# Autodesk Inventor assembly: Turnigy SK8 5045 (IGES V1)
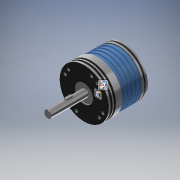
[picture p0: Inventor's stored thumbnail of the model, 180x180]
Saved by Autodesk Inventor 2019.2 (Build 232265000, 265)
## iProperties
Company: unknown
Created: 2018-11-25
Part Number: Turnigy SK8 5045 (IGES V1)
Document SubType Name: Assembly
Designer: Petar
Sending System: unknown
Preprocessor: unknown
Minimum Resolution: 0.01
Sending System Product ID: Turnigy SK8 5045 (IGES V1)
Sent Units: Millimeter
Translation Standard: IGES 5.3
Model Creation Time: 2018-11-25
Title: Turnigy SK8 5045 (IGES V1)
Author: emisnug
## Documents named in this file (8)
- D:\OMG\E-Board\CAD\Inventor\Electric Motor\Turnigy SK8 5045 (IGES V1).iam
- D:\OMG\E-Board\CAD\Inventor\Electric Motor\Magnets v9.ipt
- D:\OMG\E-Board\CAD\Inventor\Electric Motor\Can v14.ipt
- D:\OMG\E-Board\CAD\Inventor\Electric Motor\Shaft v2.ipt
- D:\OMG\E-Board\CAD\Inventor\Electric Motor\Stator Core v1.ipt
- D:\OMG\E-Board\CAD\Inventor\Electric Motor\Front Part v5.ipt
- D:\OMG\E-Board\CAD\Inventor\Electric Motor\Bearing (False - Needs Updating) v1.ipt
- D:\OMG\E-Board\CAD\Inventor\Electric Motor\feather_key.ipt
## Components (7 placed, 7 different names)
1. Magnets v9:1 — Mate:1, Mate:3, Mate:4, Mate:5, Flush:1
2. Shaft v2:1 — Rigid:1, Rigid:3
3. Stator Core v1:1 — Mate:1, Flush:1
4. Front Part v5:1 — Mate:2, Insert:1, Rigid:4
5. Bearing (False - Needs Updating) v1:1 — Mate:2, Insert:1
6. Can v14:1 — Mate:3, Mate:4, Mate:5, Rigid:1, Rigid:4
7. feather_key:1 — Rigid:3
## Relationships (10: Mate 5, WeldJoint 3, Insert 1, Flush 1)
- Mate:1: Magnets v9:1 ↔ Stator Core v1:1
- Mate:2: Front Part v5:1 ↔ Bearing (False - Needs Updating) v1:1
- Insert:1: Front Part v5:1 ↔ Bearing (False - Needs Updating) v1:1
- Mate:3: Magnets v9:1 ↔ Can v14:1
- Mate:4: Magnets v9:1 ↔ Can v14:1
- Mate:5: Magnets v9:1 ↔ Can v14:1
- Flush:1: Magnets v9:1 ↔ Stator Core v1:1
- Rigid:1 [WeldJoint]: Shaft v2:1 ↔ Can v14:1
- Rigid:3 [WeldJoint]: Shaft v2:1 ↔ feather_key:1
- Rigid:4 [WeldJoint]: Front Part v5:1 ↔ Can v14:1
